# Autodesk Inventor assembly: Torretta
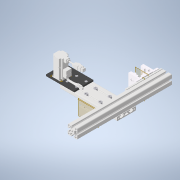
[picture p0: Inventor's stored thumbnail of the model, 180x180]
Saved by Autodesk Inventor 2022 (Build 260153000, 153)
## iProperties
Created: 2022-01-06
Part Number: Torretta
Document SubType Name: Assembly
Designer: matte
Author: matte
## Documents named in this file (15)
- C:\Users\Elia\Documents\ELIA\UNITN\MAGISTRALE\1st year\1st semester\Mechanical Design\MDM-CyberOrto-CAD\Torretta.iam
- C:\Users\Elia\Documents\ELIA\UNITN\MAGISTRALE\1st year\1st semester\Mechanical Design\MDM-CyberOrto-CAD\Carrello.iam
- C:\Users\Elia\Documents\ELIA\UNITN\MAGISTRALE\1st year\1st semester\Mechanical Design\MDM-CyberOrto-CAD\Parker components\08-Linear Application\01-Double Flange Slide Blocks\03-Metric Slide Blocks\30-4001.ipt
- C:\Users\Elia\Documents\ELIA\UNITN\MAGISTRALE\1st year\1st semester\Mechanical Design\MDM-CyberOrto-CAD\Parker components\03-Brackets_Gussets_Plates\07-Joining Plates\20-112.ipt
- C:\Users\Elia\Documents\ELIA\UNITN\MAGISTRALE\1st year\1st semester\Mechanical Design\MDM-CyberOrto-CAD\Pezzi singoli\Torretta\10-040.ipt
- C:\Users\Elia\Documents\ELIA\UNITN\MAGISTRALE\1st year\1st semester\Mechanical Design\MDM-CyberOrto-CAD\Parker components\02-Fasteners\10-Standard T-Nuts\20-058.ipt
- C:\Users\Elia\Documents\ELIA\UNITN\MAGISTRALE\1st year\1st semester\Mechanical Design\MDM-CyberOrto-CAD\Parker components\02-Fasteners\16-Screws\01-Metric Screws\01-Button Head\24-125-8.ipt
- C:\Users\Elia\Documents\ELIA\UNITN\MAGISTRALE\1st year\1st semester\Mechanical Design\MDM-CyberOrto-CAD\Parker components\02-Fasteners\10-Standard T-Nuts\20-050.ipt
- C:\Users\Elia\Documents\ELIA\UNITN\MAGISTRALE\1st year\1st semester\Mechanical Design\MDM-CyberOrto-CAD\Platform.ipt
- C:\Users\Elia\Documents\ELIA\UNITN\MAGISTRALE\1st year\1st semester\Mechanical Design\MDM-CyberOrto-CAD\Parker components\02-Fasteners\16-Screws\01-Metric Screws\01-Button Head\24-130-6.ipt
- C:\Users\Elia\Documents\ELIA\UNITN\MAGISTRALE\1st year\1st semester\Mechanical Design\MDM-CyberOrto-CAD\Parker components\02-Fasteners\15-T-Bolts_Nuts_Washers\03-Washers\24-700-6.ipt
- C:\Users\Elia\Documents\ELIA\UNITN\MAGISTRALE\1st year\1st semester\Mechanical Design\MDM-CyberOrto-CAD\Parker components\02-Fasteners\15-T-Bolts_Nuts_Washers\02-Nuts\24-706-6.ipt
- C:\Users\Elia\Documents\ELIA\UNITN\MAGISTRALE\1st year\1st semester\Mechanical Design\MDM-CyberOrto-CAD\Servo Motor 50W\bch2mba531ca5c.ipt
- C:\Users\Elia\Documents\ELIA\UNITN\MAGISTRALE\1st year\1st semester\Mechanical Design\MDM-CyberOrto-CAD\Inventor Support\Content Center Files\it-IT\ISO 1580\ISO 1580 - M4 x 12_.ipt
- C:\Users\Elia\Documents\ELIA\UNITN\MAGISTRALE\1st year\1st semester\Mechanical Design\MDM-CyberOrto-CAD\Inventor Support\Content Center Files\it-IT\AS 1474(1)\AS 1474 - M4(1).ipt
## Components (33 placed, 14 different names)
1. Carrello:1 [sub-assembly] — Coincidente:1, Coincidente:14, Allineato:8, Angolo:3, Tangente:1, Allineato:9, Coincidente:18, Allineato:12, Coincidente:43, Coincidente:44, Coincidente:45, Coincidente:46, Coincidente:47, Coincidente:48
2. 10-040:1 — Coincidente:1, Allineato:6, Coincidente:5, Allineato:7, Angolo:1, Coincidente:7, Coincidente:12, Allineato:8, Coincidente:15, Angolo:4, Allineato:11
3. 20-050:1 — Coincidente:15, Angolo:4, Allineato:9, Coincidente:16, Coincidente:17, Allineato:11
4. 24-125-8:3 — Coincidente:16, Allineato:10, Coincidente:18
5. 24-125-8:4 — Coincidente:17, Allineato:10
6. Platform:1 — Allineato:12, Coincidente:43, Coincidente:44
7. 24-130-6:1
8. 24-700-6:1
9. 24-706-6:1 — Coincidente:45
10. 24-130-6:2
11. 24-700-6:2
12. 24-130-6:3
13. 24-700-6:3
14. 24-130-6:4
15. 24-700-6:4
16. 24-706-6:2 — Coincidente:46
17. 24-706-6:3 — Coincidente:48
18. 24-706-6:4 — Coincidente:47
19. bch2mba531ca5c:1
20. ISO 1580 M4 x 12:1
21. AS 1474 - Metrico M4:1
22. ISO 1580 M4 x 12:2
23. AS 1474 - Metrico M4:2
24. AS 1474 - Metrico M4:3
25. AS 1474 - Metrico M4:4
26. ISO 1580 M4 x 12:3
27. ISO 1580 M4 x 12:4
28. 30-4001:1 — Coincidente:2, Coincidente:3, Coincidente:4, Coincidente:6, Coincidente:13
29. 20-112:1 — Coincidente:2, Coincidente:3, Coincidente:4, Allineato:6, Coincidente:5, Allineato:7, Coincidente:8, Coincidente:9, Coincidente:10, Coincidente:14
30. 20-058:1 — Angolo:1, Angolo:2, Coincidente:11, Coincidente:12
31. 24-125-8:1 — Coincidente:6, Coincidente:11, Coincidente:13
32. 20-058:2 — Angolo:2, Coincidente:7, Coincidente:8
33. 24-125-8:2 — Coincidente:9, Coincidente:10
## Relationships (67: Mate 47, Insert 8, Flush 7, Angle 4, Tangent 1)
- Coincidente:1 [Mate]: Carrello:1 ↔ 10-040:1
- Coincidente:2 [Mate]: 30-4001:1 ↔ 20-112:1
- Coincidente:3 [Mate]: 30-4001:1 ↔ 20-112:1
- Coincidente:4 [Mate]: 30-4001:1 ↔ 20-112:1
- Allineato:6 [Flush]: 10-040:1 ↔ 20-112:1
- Coincidente:5 [Mate]: 10-040:1 ↔ 20-112:1
- Allineato:7 [Flush]: 10-040:1 ↔ 20-112:1
- Coincidente:6 [Mate]: 30-4001:1 ↔ 24-125-8:1
- Angolo:1 [Angle] (180 deg): 10-040:1 ↔ 20-058:1
- Angolo:2 [Angle] (180 deg): 20-058:1 ↔ 20-058:2
- Coincidente:7 [Mate]: 10-040:1 ↔ 20-058:2
- Coincidente:8 [Mate]: 20-112:1 ↔ 20-058:2
- Coincidente:9 [Mate]: 20-112:1 ↔ 24-125-8:2
- Coincidente:10 [Mate]: 20-112:1 ↔ 24-125-8:2
- Coincidente:11 [Mate]: 20-058:1 ↔ 24-125-8:1
- Coincidente:12 [Mate]: 10-040:1 ↔ 20-058:1
- Coincidente:13 [Mate]: 30-4001:1 ↔ 24-125-8:1
- Coincidente:14 [Mate]: Carrello:1 ↔ 20-112:1
- Allineato:8 [Flush]: Carrello:1 ↔ 10-040:1
- Angolo:3 [Angle] (0 deg): Carrello:1
- Tangente:1: Carrello:1
- Coincidente:15 [Mate]: 10-040:1 ↔ 20-050:1
- Angolo:4 [Angle] (0 deg): 10-040:1 ↔ 20-050:1
- Allineato:9 [Flush] (-12.5 mm): Carrello:1 ↔ 20-050:1
- Coincidente:16 [Mate]: 20-050:1 ↔ 24-125-8:3
- Coincidente:17 [Mate]: 20-050:1 ↔ 24-125-8:4
- Allineato:10 [Flush]: 24-125-8:3 ↔ 24-125-8:4
- Coincidente:18 [Mate]: Carrello:1 ↔ 24-125-8:3
- Allineato:11 [Flush] (20 mm): 10-040:1 ↔ 20-050:1
- [Insert]: 24-130-6:1 ↔ 24-700-6:1
- [Insert]: 24-130-6:2 ↔ 24-700-6:2
- [Insert]: 24-130-6:3 ↔ 24-700-6:3
- [Insert]: 24-130-6:4 ↔ 24-700-6:4
- [Insert]: Platform:1 ↔ 24-700-6:4
- [Insert]: Platform:1 ↔ 24-700-6:3
- [Insert]: Platform:1 ↔ 24-700-6:1
- [Insert]: Platform:1 ↔ 24-700-6:2
- [Mate]: 24-130-6:2 ↔ 24-706-6:3
- [Mate]: 24-130-6:1 ↔ 24-706-6:4
- [Mate]: 24-130-6:3 ↔ 24-706-6:2
- [Mate]: 24-706-6:1 ↔ 24-130-6:4
- [Mate]: bch2mba531ca5c:1 ↔ ISO 1580 M4 x 12:1
- [Mate]: ISO 1580 M4 x 12:1 ↔ AS 1474 - Metrico M4:1
- [Mate]: bch2mba531ca5c:1 ↔ ISO 1580 M4 x 12:4
- [Mate]: bch2mba531ca5c:1 ↔ ISO 1580 M4 x 12:4
- [Mate]: AS 1474 - Metrico M4:2 ↔ ISO 1580 M4 x 12:4
- [Mate]: bch2mba531ca5c:1 ↔ ISO 1580 M4 x 12:3
- [Mate]: bch2mba531ca5c:1 ↔ ISO 1580 M4 x 12:3
- [Mate]: bch2mba531ca5c:1 ↔ ISO 1580 M4 x 12:2
- [Mate]: bch2mba531ca5c:1 ↔ ISO 1580 M4 x 12:2
- [Mate]: Platform:1 ↔ bch2mba531ca5c:1
- [Mate]: Platform:1 ↔ ISO 1580 M4 x 12:2
- [Mate]: Platform:1 ↔ ISO 1580 M4 x 12:4
- [Mate]: bch2mba531ca5c:1 ↔ ISO 1580 M4 x 12:1
- [Mate]: ISO 1580 M4 x 12:2 ↔ AS 1474 - Metrico M4:4
- [Mate]: Platform:1 ↔ AS 1474 - Metrico M4:4
- [Mate]: AS 1474 - Metrico M4:3 ↔ ISO 1580 M4 x 12:3
- [Mate]: Platform:1 ↔ AS 1474 - Metrico M4:3
- [Mate]: Platform:1 ↔ AS 1474 - Metrico M4:1
- [Mate]: Platform:1 ↔ AS 1474 - Metrico M4:2
- Allineato:12 [Flush]: Carrello:1 ↔ Platform:1
- Coincidente:43 [Mate]: Carrello:1 ↔ Platform:1
- Coincidente:44 [Mate] (-60 mm): Carrello:1 ↔ Platform:1
- Coincidente:45 [Mate]: Carrello:1 ↔ 24-706-6:1
- Coincidente:46 [Mate]: Carrello:1 ↔ 24-706-6:2
- Coincidente:47 [Mate]: Carrello:1 ↔ 24-706-6:4
- Coincidente:48 [Mate]: Carrello:1 ↔ 24-706-6:3
## Named parameters: d464_d326 = 0 mm, d465_d328 = 0 mm, d466_d330 = 0 mm, d467_d332 = 0 mm, d468_d333_d234 = 0 mm, d469_d334_d235 = 0 mm, d470_d335_d237 = 0 mm, d471_d336_d238 = 0 mm, d472_d337_d239 = 0 mm, d473_d338_d241 = 0 mm, d474_d339_d242 = 0 mm, d475_d341_d245 = 0 mm, d476_d342_d246 = 0 mm, d477_d344 = 0 mm, d478_d345 = 0 mm, d479_d346 = 0 mm, d480_d347 = 0 mm, d481_d349 = 0 mm, d482_d350 = 0 mm, d483_d351 = 0 mm, d484_d352 = 0 mm, d485_d353 = 0 mm, d486_d354 = 0 mm, d487_d311_d115 = 0 mm, d488_d312_d116_d115 = 0 mm, d489_d313_d117_d115 = 0 mm, d490_d314_d118_d115 = 0 mm, d491_d315_d119 = 0 mm, d492_d316_d120 = 0 mm, d493_d317_d121 = 0 mm, d494_d318_d122 = 0 mm
